# Autodesk Inventor assembly: Turret_Assem
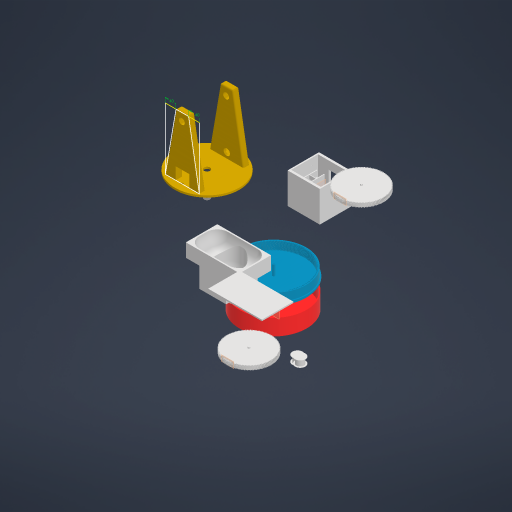
[picture p0: Inventor's stored thumbnail of the model, 512x512]
Saved by Autodesk Inventor 2023 (Build 270158000, 158)
## iProperties
Created: 2022-05-13
Part Number: Turret_Assem
Document SubType Name: Assembly
Designer: jayso
Author: jayso
## Documents named in this file (12)
- C:\Users\jayso\Desktop\Turret_CAD\CAD\Turret_Assem.iam
- C:\Users\jayso\Desktop\Turret_CAD\CAD\electronics-base.ipt
- C:\Users\jayso\Desktop\Turret_CAD\CAD\electronics-cover.ipt
- C:\Users\jayso\Desktop\Turret_CAD\CAD\y-axis-gear.ipt
- C:\Users\jayso\Desktop\Turret_CAD\CAD\x-axis-gear.ipt
- C:\Users\jayso\Desktop\Turret_CAD\CAD\turret-base.ipt
- C:\Users\jayso\Desktop\Turret_CAD\CAD\shooter-comp.ipt
- C:\Users\jayso\Desktop\Turret_CAD\CAD\shooter-right-shaft-attach.ipt
- C:\Users\jayso\Desktop\Turret_CAD\CAD\clip.ipt
- C:\Users\jayso\Desktop\Turret_CAD\CAD\clip-cover.ipt
- C:\Users\jayso\Desktop\Turret_CAD\CAD\flywheels.ipt
- C:\Users\jayso\Desktop\Turret_CAD\CAD\Turret_Assem\Design Accelerator\Bearing1.iam
## Components (13 placed, 11 different names)
1. electronics-base:1
2. electronics-cover:1
3. y-axis-gear:1
4. x-axis-gear:1
5. turret-base:1 — Mate:1
6. shooter-comp:1
7. shooter-right-shaft-attach:1
8. clip:1
9. clip-cover:1
10. flywheels:1
11. shooter-right-shaft-attach:2
12. flywheels:2
13. Bearing:1 [sub-assembly] — Mate:1
## Relationships (1: Mate 1)
- Mate:1: turret-base:1 ↔ Bearing:1
